# Autodesk Inventor assembly: gyroPhone01
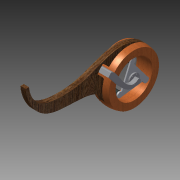
[picture p0: Inventor's stored thumbnail of the model, 180x180]
Saved by Autodesk Inventor 2013 (Build 170138000, 138)
## iProperties
Created: 2013-01-08
Part Number: gyroPhone01
Document SubType Name: Assembly
Designer: Nano
Author: Nano
## Documents named in this file (7)
- C:\Users\Nano\Documents\InventorByron\InventorMasterProject\gyroPhone01\gyroPhone01.iam
- C:\Users\Nano\Documents\InventorByron\InventorMasterProject\gyroPhone01\bodySphere.ipt
- C:\Users\Nano\Documents\InventorByron\InventorMasterProject\gyroPhone01\bigWheel.ipt
- C:\Users\Nano\Documents\InventorByron\InventorMasterProject\gyroPhone01\bodyMainAirPipe.ipt
- C:\Users\Nano\Documents\InventorByron\InventorMasterProject\gyroPhone01\motorAssembly01.iam
- C:\Users\Nano\Documents\InventorByron\InventorMasterProject\gyroPhone01\motorPlate.ipt
- C:\Users\Nano\Documents\InventorByron\InventorMasterProject\gyroPhone01\fork.ipt
## Components (8 placed, 6 different names)
1. bodySphere:1
2. bigWheel:1 — Tangent:1, Flush:2
3. bodyMainAirPipe:1 — Flush:1
4. motorPlate:1 — Flush:3, Mate:1, Mate:2, Mate:3, Mate:4
5. fork:1 — Mate:1
6. motorAssembly01:1 [sub-assembly] — Tangent:1, Flush:2, Mate:3
7. motorAssembly01:2 [sub-assembly] — Flush:3, Mate:4
8. motorAssembly01:3 [sub-assembly] — Mate:2
## Component patterns: (3 elements, first: motorAssembly01:1)
## Relationships (8: Mate 4, Flush 3, Tangent 1)
- Flush:1: bodyMainAirPipe:1
- Tangent:1: bigWheel:1 ↔ motorAssembly01:1
- Flush:2 (38.1 mm): bigWheel:1 ↔ motorAssembly01:1
- Flush:3: motorPlate:1 ↔ motorAssembly01:2
- Mate:1: motorPlate:1 ↔ fork:1
- Mate:2: motorPlate:1 ↔ motorAssembly01:3
- Mate:3: motorPlate:1 ↔ motorAssembly01:1
- Mate:4: motorPlate:1 ↔ motorAssembly01:2
